# Autodesk Inventor assembly: dash_v3
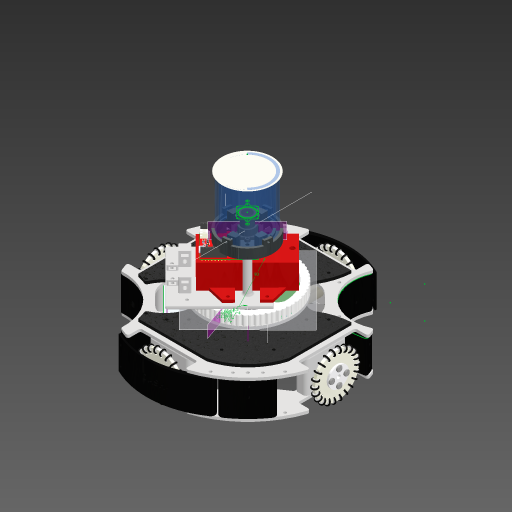
[picture p0: Inventor's stored thumbnail of the model, 512x512]
Saved by Autodesk Inventor 2023 (Build 270158000, 158)
## iProperties
Created: 2025-08-06
Part Number: dash_v3
Document SubType Name: Assembly
Designer: daa
Author: daa
## Documents named in this file (5)
- C:\Users\daa\Documents\DASH_V2\dash_v3.iam
- C:\Users\daa\Documents\DASH_V2\omni_platforma\omni_platformaV2.iam
- C:\Users\daa\Documents\DASH_V2\tower_V2.iam
- C:\Users\daa\Documents\DASH_V2\rack_25.ipt
- C:\Users\daa\Documents\DASH_V2\boost converter 50V.ipt
## Components (7 placed, 4 different names)
1. omni_platformaV2:1 [sub-assembly] — Совмещение:2, Совмещение:3, Совмещение:4, Совмещение:5, С поворотом:2
2. tower_V2:1 [sub-assembly] — Совмещение:6, С поворотом:1
3. rack_25:1 — Совмещение:2, Совмещение:6
4. rack_25:2 — Совмещение:4
5. rack_25:3 — Совмещение:3, С поворотом:1
6. rack_25:4 — Совмещение:5
7. boost converter 50V:1 — С поворотом:2
## Relationships (7: Mate 5, RevoluteJoint 2)
- Совмещение:2 [Mate]: omni_platformaV2:1 ↔ rack_25:1
- Совмещение:3 [Mate]: omni_platformaV2:1 ↔ rack_25:3
- Совмещение:4 [Mate]: omni_platformaV2:1 ↔ rack_25:2
- Совмещение:5 [Mate]: omni_platformaV2:1 ↔ rack_25:4
- Совмещение:6 [Mate]: tower_V2:1 ↔ rack_25:1
- С поворотом:1 [RevoluteJoint]: tower_V2:1 ↔ rack_25:3
- С поворотом:2 [RevoluteJoint]: omni_platformaV2:1 ↔ boost converter 50V:1
